# Autodesk Inventor assembly: CO-0-01-controlsBox
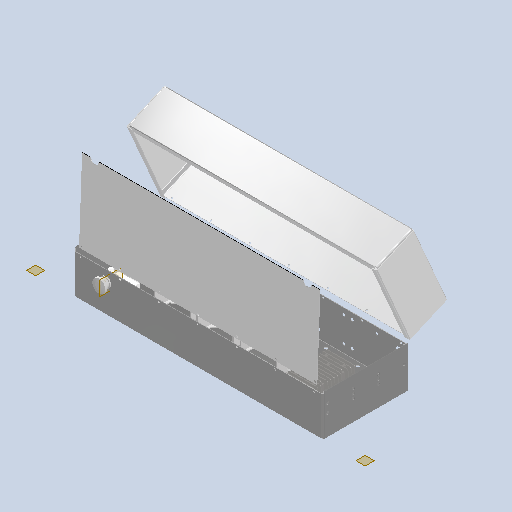
[picture p0: Inventor's stored thumbnail of the model, 512x512]
Saved by Autodesk Inventor 2025.1 (Build 291241020, 241B)
## iProperties
Created: 2023-04-11
Part Number: CO-0-01-controlsBox
Document SubType Name: Weldment
Designer: t205b
Weld Material: Welded Aluminum-6061
Author: t205b
## Documents named in this file (9)
- C:\Users\t205b\OneDrive\Documents\Github\BehrendURCMechanical\CAD\Controls\Protocase Controls Box\CO-0-03-controlsBox.iam
- C:\Users\t205b\OneDrive\Documents\Github\BehrendURCMechanical\CAD\Controls\Protocase Controls Box\CO-1-07-controlsBox.ipt
- C:\Users\t205b\OneDrive\Documents\Github\BehrendURCMechanical\CAD\Controls\Protocase Controls Box\CO-1-04-controlsSeperator.ipt
- C:\Users\t205b\OneDrive\Documents\Github\BehrendURCMechanical\CAD\Controls\Protocase Controls Box\CO-1-04-controlsLid.ipt
- C:\Users\t205b\OneDrive\Documents\Github\BehrendURCMechanical\CAD\Controls\CO-1-01-voltageRegulator.ipt
- C:\Users\t205b\OneDrive\Documents\Github\BehrendURCMechanical\CAD\Controls\CO-1-06-fuseMountBottom.ipt
- C:\Users\t205b\OneDrive\Documents\Github\BehrendURCMechanical\CAD\Controls\CO-1-02-relay.ipt
- C:\Users\t205b\OneDrive\Documents\Github\BehrendURCMechanical\CAD\Controls\CO-1-01-eStopButton.ipt
- C:\Users\t205b\OneDrive\Documents\Github\BehrendURCMechanical\CAD\Controls\CO-1-01-circuitBreaker250a.ipt
## Components (10 placed, 8 different names)
1. CO-1-07-controlsBox:1 — Cylindrical:1, Flush:1, Cylindrical:2, Mate:1, Mate:2, Mate:5, Mate:6, Mate:7, Mate:8, Mate:9, Mate:10, Mate:12, Insert:1, Insert:2, Insert:3, Mate:13, Insert:4, Mate:14, Insert:5, Insert:6, Insert:7, Mate:15
2. CO-1-04-controlsSeperator:1 — Cylindrical:2, Mate:1
3. CO-1-04-controlsLid:1 — Cylindrical:1, Flush:1
4. CO-1-06-fuseMountBottom:1 — Mate:9, Mate:10
5. CO-1-06-fuseMountBottom:2 — Mate:7, Mate:8
6. CO-1-06-fuseMountBottom:3 — Mate:5, Mate:6
7. CO-1-01-eStopButton:1 — Insert:7, Mate:15
8. CO-1-01-circuitBreaker250a:1 — Mate:12, Insert:1, Insert:2, Insert:3
9. CO-1-02-relay:1 — Mate:13, Insert:4
10. CO-1-01-voltageRegulator:1 — Mate:14, Insert:5, Insert:6
## Relationships (22: Mate 12, Insert 7, CylindricalJoint 2, Flush 1)
- Cylindrical:1: CO-1-07-controlsBox:1 ↔ CO-1-04-controlsLid:1
- Flush:1: CO-1-07-controlsBox:1 ↔ CO-1-04-controlsLid:1
- Cylindrical:2: CO-1-07-controlsBox:1 ↔ CO-1-04-controlsSeperator:1
- Mate:1: CO-1-07-controlsBox:1 ↔ CO-1-04-controlsSeperator:1
- Mate:2: CO-1-07-controlsBox:1
- Mate:5: CO-1-07-controlsBox:1 ↔ CO-1-06-fuseMountBottom:3
- Mate:6: CO-1-07-controlsBox:1 ↔ CO-1-06-fuseMountBottom:3
- Mate:7: CO-1-07-controlsBox:1 ↔ CO-1-06-fuseMountBottom:2
- Mate:8: CO-1-07-controlsBox:1 ↔ CO-1-06-fuseMountBottom:2
- Mate:9: CO-1-07-controlsBox:1 ↔ CO-1-06-fuseMountBottom:1
- Mate:10: CO-1-07-controlsBox:1 ↔ CO-1-06-fuseMountBottom:1
- Mate:12: CO-1-07-controlsBox:1 ↔ CO-1-01-circuitBreaker250a:1
- Insert:1: CO-1-07-controlsBox:1 ↔ CO-1-01-circuitBreaker250a:1
- Insert:2: CO-1-07-controlsBox:1 ↔ CO-1-01-circuitBreaker250a:1
- Insert:3: CO-1-07-controlsBox:1 ↔ CO-1-01-circuitBreaker250a:1
- Mate:13: CO-1-07-controlsBox:1 ↔ CO-1-02-relay:1
- Insert:4: CO-1-07-controlsBox:1 ↔ CO-1-02-relay:1
- Mate:14: CO-1-07-controlsBox:1 ↔ CO-1-01-voltageRegulator:1
- Insert:5: CO-1-07-controlsBox:1 ↔ CO-1-01-voltageRegulator:1
- Insert:6: CO-1-07-controlsBox:1 ↔ CO-1-01-voltageRegulator:1
- Insert:7: CO-1-07-controlsBox:1 ↔ CO-1-01-eStopButton:1
- Mate:15: CO-1-07-controlsBox:1 ↔ CO-1-01-eStopButton:1
